# Autodesk Inventor assembly: ensamble caja motriz
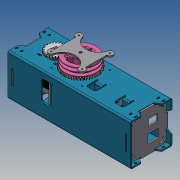
[picture p0: Inventor's stored thumbnail of the model, 180x180]
Saved by Autodesk Inventor 2017 (Build 210142000, 142)
## iProperties
Part Number: ensamble caja motriz
Material: Genérico
Document SubType Name: Assembly
Designer: leo
Author: FABLAB
## Documents named in this file (8)
- C:\Users\Leo\Documents\GitHub\actor-re-actor\models\inventor-caja\ensamble caja motriz.iam
- C:\Users\Leo\Documents\GitHub\actor-re-actor\models\inventor-caja\transmision Engranajes\Potencia.iam
- C:\Users\Leo\Documents\GitHub\actor-re-actor\models\inventor-caja\transmision Engranajes\conjunto plato-carrete.iam
- C:\Users\Leo\Documents\GitHub\actor-re-actor\models\inventor-caja\ensamble caja motriz\Design Accelerator\Engranajes rectos1.iam
- C:\Users\Leo\Documents\GitHub\actor-re-actor\models\inventor-caja\ensamble caja motriz\Design Accelerator\Conexión por perno1.iam
- C:\Users\Leo\Documents\GitHub\actor-re-actor\models\inventor-caja\ensamble caja motriz\Design Accelerator\Conexión por perno2.iam
- C:\Users\Leo\Documents\GitHub\actor-re-actor\models\inventor-caja\Piezas\componentes.iam
- C:\Users\Leo\Documents\GitHub\actor-re-actor\models\inventor-caja\Case\Case-D.iam
## Components (7 placed, 6 different names)
1. Case-D:1 [sub-assembly] — Coincidencia:1, Coincidencia:4, Coincidencia:9, Nivelación:12, Coincidencia:11, Coincidencia:12, Coincidencia:13
2. Potencia:1 [sub-assembly] — Coincidencia:1, Coincidencia:2, Coincidencia:3, Coincidencia:10
3. conjunto plato-carrete:1 [sub-assembly] — Coincidencia:4, Coincidencia:5, Coincidencia:6
4. Engranajes rectos:1 [sub-assembly]
5. Conexión por perno:1 [sub-assembly] — Coincidencia:12, Coincidencia:13
6. Conexión por perno:2 [sub-assembly] — Coincidencia:9, Coincidencia:10
7. componentes:1 [sub-assembly] — Nivelación:12, Coincidencia:11
## Relationships (12: Mate 11, Flush 1)
- Coincidencia:1 [Mate]: Case-D:1 ↔ Potencia:1
- Coincidencia:2 [Mate]: Potencia:1
- Coincidencia:3 [Mate]: Potencia:1
- Coincidencia:4 [Mate] (5 mm): Case-D:1 ↔ conjunto plato-carrete:1
- Coincidencia:5 [Mate]: conjunto plato-carrete:1
- Coincidencia:6 [Mate] (72 mm): conjunto plato-carrete:1
- Coincidencia:9 [Mate]: Case-D:1 ↔ Conexión por perno:2
- Coincidencia:10 [Mate]: Potencia:1 ↔ Conexión por perno:2
- Nivelación:12 [Flush]: Case-D:1 ↔ componentes:1
- Coincidencia:11 [Mate]: Case-D:1 ↔ componentes:1
- Coincidencia:12 [Mate]: Case-D:1 ↔ Conexión por perno:1
- Coincidencia:13 [Mate]: Case-D:1 ↔ Conexión por perno:1
